# Autodesk Inventor assembly: 217-3268-3CIM_WCD_orient2
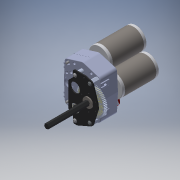
[picture p0: Inventor's stored thumbnail of the model, 180x180]
Saved by Autodesk Inventor 2016 (Build 200138000, 138)
## iProperties
Created: 2015-12-17
Part Number: 217-3268-3CIM_WCD_orient2
Description: STEP AP214
Document SubType Name: Assembly
Designer: rickab1
Sending System: SolidWorks 2015
Preprocessor: SwSTEP 2.0
Title: 217-3268-STEP-20151217.STEP
Revision Number: ANY
## Documents named in this file (56)
- C:\Users\rickab1\Documents\Inventor\gearboxes\3CIM BS 3rd Stage\217-3268-STEP-20151217v2\217-3268-3CIM_WCD_orient2.iam
- C:\Users\rickab1\Documents\Inventor\gearboxes\3CIM BS 3rd Stage\217-3268-STEP-20151217v2\217-2733-001 Rev2.ipt
- C:\Users\rickab1\Documents\Inventor\gearboxes\3CIM BS 3rd Stage\217-3268-STEP-20151217v2\217-2731-001 Rev2.ipt
- C:\Users\rickab1\Documents\Inventor\gearboxes\3CIM BS 3rd Stage\217-3268-STEP-20151217v2\217-2789-001 Rev2.ipt
- C:\Users\rickab1\Documents\Inventor\gearboxes\3CIM BS 3rd Stage\217-3268-STEP-20151217v2\217-2778-001 Rev2_NCQ8A075-050M.iam
- C:\Users\rickab1\Documents\Inventor\gearboxes\3CIM BS 3rd Stage\217-3268-STEP-20151217v2\217-2428-012 Rev2.ipt
- C:\Users\rickab1\Documents\Inventor\gearboxes\3CIM BS 3rd Stage\217-3268-STEP-20151217v2\217-2428-005 Rev1.ipt
- C:\Users\rickab1\Documents\Inventor\gearboxes\3CIM BS 3rd Stage\217-3268-STEP-20151217v2\SCREW-832-0375.ipt
- C:\Users\rickab1\Documents\Inventor\gearboxes\3CIM BS 3rd Stage\217-3268-STEP-20151217v2\SBS1_SBS-0632-0250.ipt
- C:\Users\rickab1\Documents\Inventor\gearboxes\3CIM BS 3rd Stage\217-3268-STEP-20151217v2\217-4098-100 Rev1.iam
- C:\Users\rickab1\Documents\Inventor\gearboxes\3CIM BS 3rd Stage\217-3268-STEP-20151217v2\217-2428-017 Rev2.ipt
- C:\Users\rickab1\Documents\Inventor\gearboxes\3CIM BS 3rd Stage\217-3268-STEP-20151217v2\217-2428-016 Rev3_Spur01.ipt
- C:\Users\rickab1\Documents\Inventor\gearboxes\3CIM BS 3rd Stage\217-3268-STEP-20151217v2\217-2428-019 Rev1.ipt
- C:\Users\rickab1\Documents\Inventor\gearboxes\3CIM BS 3rd Stage\217-3268-STEP-20151217v2\217-2428-006 Rev1.ipt
- C:\Users\rickab1\Documents\Inventor\gearboxes\3CIM BS 3rd Stage\217-3268-STEP-20151217v2\217-2614-001_12t.ipt
- C:\Users\rickab1\Documents\Inventor\gearboxes\3CIM BS 3rd Stage\217-3268-STEP-20151217v2\217-2761-001 rev1.ipt
- C:\Users\rickab1\Documents\Inventor\gearboxes\3CIM BS 3rd Stage\217-3268-STEP-20151217v2\217-3195-002 rev2.ipt
- C:\Users\rickab1\Documents\Inventor\gearboxes\3CIM BS 3rd Stage\217-3268-STEP-20151217v2\217-3195-001 Rev1.ipt
- C:\Users\rickab1\Documents\Inventor\gearboxes\3CIM BS 3rd Stage\217-3268-STEP-20151217v2\276-1027-001.ipt
- C:\Users\rickab1\Documents\Inventor\gearboxes\3CIM BS 3rd Stage\217-3268-STEP-20151217v2\SCREW-832-1750.ipt
- C:\Users\rickab1\Documents\Inventor\gearboxes\3CIM BS 3rd Stage\217-3268-STEP-20151217v2\217-2428-004 Rev3.ipt
- C:\Users\rickab1\Documents\Inventor\gearboxes\3CIM BS 3rd Stage\217-3268-STEP-20151217v2\217-2428-021 Rev1.ipt
- C:\Users\rickab1\Documents\Inventor\gearboxes\3CIM BS 3rd Stage\217-3268-STEP-20151217v2\217-2428-029 Rev1.ipt
- C:\Users\rickab1\Documents\Inventor\gearboxes\3CIM BS 3rd Stage\217-3268-STEP-20151217v2\Grayhill Lock Washer.ipt
- C:\Users\rickab1\Documents\Inventor\gearboxes\3CIM BS 3rd Stage\217-3268-STEP-20151217v2\Grayhill Nut.ipt
- C:\Users\rickab1\Documents\Inventor\gearboxes\3CIM BS 3rd Stage\217-3268-STEP-20151217v2\217-2000.ipt
- C:\Users\rickab1\Documents\Inventor\gearboxes\3CIM BS 3rd Stage\217-3268-STEP-20151217v2\Grahill Encoder.ipt
- C:\Users\rickab1\Documents\Inventor\gearboxes\3CIM BS 3rd Stage\217-3268-STEP-20151217v2\SBS1_SBS-2520-125.ipt
- C:\Users\rickab1\Documents\Inventor\gearboxes\3CIM BS 3rd Stage\217-3268-STEP-20151217v2\217-3195-008 Rev1_stubby .75_.ipt
- C:\Users\rickab1\Documents\Inventor\gearboxes\3CIM BS 3rd Stage\217-3268-STEP-20151217v2\Nylock Nut_NNY2520-ZC.ipt
- C:\Users\rickab1\Documents\Inventor\gearboxes\3CIM BS 3rd Stage\217-3268-STEP-20151217v2\SBS1_SBS2520-0625ZC.ipt
- C:\Users\rickab1\Documents\Inventor\gearboxes\3CIM BS 3rd Stage\217-3268-STEP-20151217v2\217-2617-002 Rev1_91780A359.ipt
- C:\Users\rickab1\Documents\Inventor\gearboxes\3CIM BS 3rd Stage\217-3268-STEP-20151217v2\217-3195-003 rev2.ipt
- C:\Users\rickab1\Documents\Inventor\gearboxes\3CIM BS 3rd Stage\217-3268-STEP-20151217v2\217-2617-003 Rev1.ipt
- C:\Users\rickab1\Documents\Inventor\gearboxes\3CIM BS 3rd Stage\217-3268-STEP-20151217v2\217-3109-001 Rev1.ipt
- C:\Users\rickab1\Documents\Inventor\gearboxes\3CIM BS 3rd Stage\217-3268-STEP-20151217v2\217-2734-001 Rev3.ipt
- C:\Users\rickab1\Documents\Inventor\gearboxes\3CIM BS 3rd Stage\217-3268-STEP-20151217v2\217-2617-004 Rev1_97431A340_grv.ipt
- C:\Users\rickab1\Documents\Inventor\gearboxes\3CIM BS 3rd Stage\217-3268-STEP-20151217v2\217-2702-001_20t.ipt
- C:\Users\rickab1\Documents\Inventor\gearboxes\3CIM BS 3rd Stage\217-3268-STEP-20151217v2\217-2715-002 Rev1_64t.ipt
- C:\Users\rickab1\Documents\Inventor\gearboxes\3CIM BS 3rd Stage\217-3268-STEP-20151217v2\217-2704-001_24.ipt
- C:\Users\rickab1\Documents\Inventor\gearboxes\3CIM BS 3rd Stage\217-3268-STEP-20151217v2\217-2714-002 Rev1_60t.ipt
- C:\Users\rickab1\Documents\Inventor\gearboxes\3CIM BS 3rd Stage\217-3268-STEP-20151217v2\217-3221-002 Rev1.ipt
- C:\Users\rickab1\Documents\Inventor\gearboxes\3CIM BS 3rd Stage\217-3268-STEP-20151217v2\217-2705-001_30t.ipt
- C:\Users\rickab1\Documents\Inventor\gearboxes\3CIM BS 3rd Stage\217-3268-STEP-20151217v2\217-2712-002 Rev1_50t.ipt
- C:\Users\rickab1\Documents\Inventor\gearboxes\3CIM BS 3rd Stage\217-3268-STEP-20151217v2\217-2706-001_34t.ipt
- C:\Users\rickab1\Documents\Inventor\gearboxes\3CIM BS 3rd Stage\217-3268-STEP-20151217v2\217-3287-001 Rev3.iam
- C:\Users\rickab1\Documents\Inventor\gearboxes\3CIM BS 3rd Stage\217-3268-STEP-20151217v2\217-3211-001 Rev1_34t.ipt
- C:\Users\rickab1\Documents\Inventor\gearboxes\3CIM BS 3rd Stage\217-3268-STEP-20151217v2\217-3288-001 Rev3.iam
- C:\Users\rickab1\Documents\Inventor\gearboxes\3CIM BS 3rd Stage\217-3268-STEP-20151217v2\217-3210-001 Rev1_30t.ipt
- C:\Users\rickab1\Documents\Inventor\gearboxes\3CIM BS 3rd Stage\217-3268-STEP-20151217v2\217-3292-001 Rev3.iam
- C:\Users\rickab1\Documents\Inventor\gearboxes\3CIM BS 3rd Stage\217-3268-STEP-20151217v2\217-2703-001.ipt
- C:\Users\rickab1\Documents\Inventor\gearboxes\3CIM BS 3rd Stage\217-3268-STEP-20151217v2\217-2711-002 Rev1_50t.ipt
- C:\Users\rickab1\Documents\Inventor\gearboxes\3CIM BS 3rd Stage\217-3268-STEP-20151217v2\217-2428-023 Rev1_9714K3.ipt
- C:\Users\rickab1\Documents\Inventor\gearboxes\3CIM BS 3rd Stage\217-3268-STEP-20151217v2\SBS_SBS2520-1750.ipt
- C:\Users\rickab1\Documents\Inventor\gearboxes\3CIM BS 3rd Stage\217-3268-STEP-20151217v2\NNYXXXX-ZZ_NNY2520-ZC.ipt
- C:\Users\rickab1\Documents\Inventor\gearboxes\3CIM BS 3rd Stage\217-3268-STEP-20151217v2\SBS_SBS2520-1500ZC.ipt
## Components (83 placed, 83 different names)
1. 217-2733-001 Rev2_1
2. 217-2733-001 Rev2_2
3. 217-2731-001 Rev2_3
4. 217-2789-001 Rev2_4
5. 217-2778-001 Rev2_NCQ8A075-050M_5 [sub-assembly]
6. 217-2428-012 Rev2_6
7. 217-2428-005 Rev1_7
8. 217-2428-005 Rev1_8
9. SCREW-832-0375_9
10. SCREW-832-0375_10
11. SCREW-832-0375_11
12. SCREW-832-0375_12
13. SBS1_SBS-0632-0250_13
14. SBS1_SBS-0632-0250_14
15. 217-4098-100 Rev1_15 [sub-assembly]
16. 217-2428-017 Rev2_16
17. 217-2428-016 Rev3_Spur01_17
18. 217-2428-019 Rev1_18
19. 217-2428-006 Rev1_19
20. 217-2428-006 Rev1_20
21. SCREW-832-0375_21
22. SCREW-832-0375_22
23. SCREW-832-0375_23
24. SCREW-832-0375_24
25. 217-2614-001_12t_25
26. 217-2761-001 rev1_26
27. 217-2761-001 rev1_27
28. 217-2614-001_12t_28
29. 217-2614-001_12t_29
30. 217-2761-001 rev1_30
31. 217-3195-002 rev2_31 — Mate:4, Mate:5, Mate:11, Mate:12, Mate:13, Mate:14
32. 217-3195-001 Rev1_32
33. 276-1027-001_33
34. 276-1027-001_34
35. SCREW-832-1750_35
36. SCREW-832-1750_36
37. 217-2428-004 Rev3_37
38. 217-2428-021 Rev1_38
39. 217-2428-029 Rev1_39
40. Grayhill Lock Washer_40
41. Grayhill Nut_41
42. 217-2000_42
43. 217-2000_43
44. 217-2000_44
45. Grahill Encoder_45
46. SBS1_SBS-2520-125_46 — Mate:7
47. 217-3195-008 Rev1_stubby .75"_47 — Mate:8
48. 217-3195-008 Rev1_stubby .75"_48
49. Nylock Nut_NNY2520-ZC_49
50. Nylock Nut_NNY2520-ZC_50
51. SBS1_SBS2520-0625ZC_51 — Mate:19, Mate:20
52. SBS1_SBS2520-0625ZC_52 — Mate:21, Mate:22
53. 217-2617-002 Rev1_91780A359_53 — Mate:4, Mate:9, Mate:12, Mate:21
54. 217-2617-002 Rev1_91780A359_54 — Mate:5, Mate:10, Mate:11
55. 217-3195-003 rev2_55 — Mate:6, Mate:7, Mate:8, Mate:9, Mate:10, Mate:19, Mate:20, Mate:22, Mate:23, Mate:24
56. 217-2617-003 Rev1_56 — Mate:15, Mate:16, Mate:17, Mate:18, Mate:25
57. 217-3109-001 Rev1_57 — Mate:13, Mate:14, Mate:17, Mate:18
58. 217-2734-001 Rev3_58 — Mate:23, Mate:24
59. 217-2617-004 Rev1_97431A340_grv_59 — Mate:15, Mate:16, Mate:26
60. 217-2617-004 Rev1_97431A340_grv_60
61. 217-2702-001_20t_61
62. 217-2715-002 Rev1_64t_62 — Mate:1, Mate:2, Flush:2
63. 217-2704-001_24_63
64. 217-2714-002 Rev1_60t_64 — Mate:1, Mate:3, Flush:3, Mate:26
65. 217-3221-002 Rev1_65 — Mate:2, Flush:1, Mate:25
66. 217-2705-001_30t_66
67. 217-2712-002 Rev1_50t_67 — Mate:3, Flush:1, Flush:2, Flush:3
68. 217-2706-001_34t_68
69. SBS1_SBS-2520-125_69 — Mate:6
70. 217-3287-001 Rev3_70 [sub-assembly]
71. 217-3211-001 Rev1_34t_71
72. 217-3288-001 Rev3_72 [sub-assembly]
73. 217-3210-001 Rev1_30t_73
74. 217-3292-001 Rev3_74 [sub-assembly]
75. 217-2703-001_75
76. 217-2711-002 Rev1_50t_76
77. 217-2428-023 Rev1_9714K3_77
78. SBS_SBS2520-1750_78
79. SBS_SBS2520-1750_79
80. NNYXXXX-ZZ_NNY2520-ZC_80
81. NNYXXXX-ZZ_NNY2520-ZC_81
82. SBS_SBS2520-1500ZC_82
83. SBS_SBS2520-1500ZC_83
## Relationships (29: Mate 26, Flush 3)
- Mate:1: 217-2715-002 Rev1_64t_62 ↔ 217-2714-002 Rev1_60t_64
- Mate:2: 217-2715-002 Rev1_64t_62 ↔ 217-3221-002 Rev1_65
- Mate:3: 217-2714-002 Rev1_60t_64 ↔ 217-2712-002 Rev1_50t_67
- Flush:1: 217-3221-002 Rev1_65 ↔ 217-2712-002 Rev1_50t_67
- Flush:2: 217-2715-002 Rev1_64t_62 ↔ 217-2712-002 Rev1_50t_67
- Flush:3: 217-2714-002 Rev1_60t_64 ↔ 217-2712-002 Rev1_50t_67
- Mate:4: 217-3195-002 rev2_31 ↔ 217-2617-002 Rev1_91780A359_53
- Mate:5: 217-3195-002 rev2_31 ↔ 217-2617-002 Rev1_91780A359_54
- Mate:6: 217-3195-003 rev2_55 ↔ SBS1_SBS-2520-125_69
- Mate:7: SBS1_SBS-2520-125_46 ↔ 217-3195-003 rev2_55
- Mate:8: 217-3195-008 Rev1_stubby .75"_47 ↔ 217-3195-003 rev2_55
- Mate:9: 217-2617-002 Rev1_91780A359_53 ↔ 217-3195-003 rev2_55
- Mate:10: 217-2617-002 Rev1_91780A359_54 ↔ 217-3195-003 rev2_55
- Mate:11: 217-3195-002 rev2_31 ↔ 217-2617-002 Rev1_91780A359_54
- Mate:12: 217-3195-002 rev2_31 ↔ 217-2617-002 Rev1_91780A359_53
- Mate:13: 217-3195-002 rev2_31 ↔ 217-3109-001 Rev1_57
- Mate:14: 217-3195-002 rev2_31 ↔ 217-3109-001 Rev1_57
- Mate:15: 217-2617-003 Rev1_56 ↔ 217-2617-004 Rev1_97431A340_grv_59
- Mate:16: 217-2617-003 Rev1_56 ↔ 217-2617-004 Rev1_97431A340_grv_59
- Mate:17: 217-2617-003 Rev1_56 ↔ 217-3109-001 Rev1_57
- Mate:18: 217-2617-003 Rev1_56 ↔ 217-3109-001 Rev1_57
- Mate:19: SBS1_SBS2520-0625ZC_51 ↔ 217-3195-003 rev2_55
- Mate:20: SBS1_SBS2520-0625ZC_51 ↔ 217-3195-003 rev2_55
- Mate:21: SBS1_SBS2520-0625ZC_52 ↔ 217-2617-002 Rev1_91780A359_53
- Mate:22: SBS1_SBS2520-0625ZC_52 ↔ 217-3195-003 rev2_55
- Mate:23: 217-3195-003 rev2_55 ↔ 217-2734-001 Rev3_58
- Mate:24: 217-3195-003 rev2_55 ↔ 217-2734-001 Rev3_58
- Mate:25: 217-2617-003 Rev1_56 ↔ 217-3221-002 Rev1_65
- Mate:26: 217-2617-004 Rev1_97431A340_grv_59 ↔ 217-2714-002 Rev1_60t_64
